# Autodesk Inventor assembly: main_assy
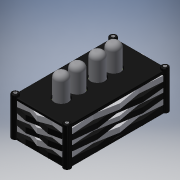
[picture p0: Inventor's stored thumbnail of the model, 180x180]
Saved by Autodesk Inventor 2017 (Build 210142000, 142)
## iProperties
Created: 2018-01-14
Part Number: main_assy
Document SubType Name: Assembly
Designer: Mitch
Author: Mitch
## Documents named in this file (26)
- E:\Youtube Channel\Pojects\Nixie Clock\Mech\main_assy.iam
- E:\Youtube Channel\Pojects\Nixie Clock\Mech\Clock Base.ipt
- E:\Youtube Channel\Pojects\Nixie Clock\Mech\PCB.ipt
- E:\Youtube Channel\Pojects\Nixie Clock\Mech\High_volt_pcb.ipt
- E:\Youtube Channel\Pojects\Nixie Clock\Mech\Case Top.ipt
- E:\Youtube Channel\Pojects\Nixie Clock\Mech\long_insert.ipt
- E:\Youtube Channel\Pojects\Nixie Clock\Mech\long_insert_inv.ipt
- E:\Youtube Channel\Pojects\Nixie Clock\Mech\Short_insert.ipt
- E:\Youtube Channel\Pojects\Nixie Clock\Mech\short_insert_invert.ipt
- E:\Youtube Channel\Pojects\Nixie Clock\Mech\long_insert_CPY.ipt
- E:\Youtube Channel\Pojects\Nixie Clock\Mech\long_insert_inv_CPY.ipt
- E:\Youtube Channel\Pojects\Nixie Clock\Mech\long_insert_CPY1.ipt
- E:\Youtube Channel\Pojects\Nixie Clock\Mech\long_insert_inv_CPY1.ipt
- E:\Youtube Channel\Pojects\Nixie Clock\Mech\Short_insert_CPY.ipt
- E:\Youtube Channel\Pojects\Nixie Clock\Mech\short_insert_invert_CPY.ipt
- E:\Youtube Channel\Pojects\Nixie Clock\Mech\Short_insert_CPY1.ipt
- E:\Youtube Channel\Pojects\Nixie Clock\Mech\short_insert_invert_CPY1.ipt
- E:\Youtube Channel\Pojects\Nixie Clock\Mech\Short_insert_CPY2.ipt
- E:\Youtube Channel\Pojects\Nixie Clock\Mech\short_insert_invert_CPY2.ipt
- E:\Youtube Channel\Pojects\Nixie Clock\Mech\Short_insert_CPY3.ipt
- E:\Youtube Channel\Pojects\Nixie Clock\Mech\short_insert_invert_CPY3.ipt
- E:\Youtube Channel\Pojects\Nixie Clock\Mech\back_plate.ipt
- E:\Youtube Channel\Pojects\Nixie Clock\Mech\91500A084_TYPE 316 SS FLAT HEAD PHILLIPS MACHINE SCREW.ipt
- E:\Youtube Channel\Pojects\Nixie Clock\Mech\Tactile switch Omron_B3F.iam
- E:\Youtube Channel\Pojects\Nixie Clock\Mech\CUI_PJ-002B.ipt
- E:\Youtube Channel\Pojects\Nixie Clock\Mech\push_buttons.ipt
## Components (31 placed, 25 different names)
1. Clock Base:1 — Mate:4, Mate:5, Mate:6, Mate:7, Mate:8, Mate:9, Mate:10, Mate:12, Mate:13, Mate:14, Mate:16, Mate:17, Mate:19, Mate:20, Mate:21, Mate:22, Mate:23, Mate:25, Mate:26, Mate:31, Mate:32, Mate:33, Mate:34, Mate:35, Mate:36, Mate:37, Mate:38, Mate:39, Mate:44, Mate:45, Mate:46, Mate:47, Mate:48, Mate:49, Mate:50, Mate:51, Mate:56, Mate:57, Mate:58, Mate:59, Mate:60, Mate:61, Mate:62, Mate:63, Mate:64, Mate:65, Mate:66, Flush:1, Mate:68, Mate:69, Mate:70, Mate:71, Mate:72
2. High_volt_pcb:1 — Mate:4, Mate:5, Mate:6
3. Case Top:1 — Mate:7, Flush:2, Flush:3, Flush:4, Flush:5
4. long_insert:1 — Mate:8, Mate:9, Mate:10, Mate:18
5. long_insert_inv:1 — Mate:18, Mate:19, Mate:20, Mate:27
6. Short_insert:1 — Mate:12, Mate:13, Mate:14, Mate:15
7. short_insert_invert:1 — Mate:15, Mate:16, Mate:17, Mate:40
8. Short_insert:2 — Mate:21, Mate:22, Mate:23, Mate:24
9. short_insert_invert:2 — Mate:24, Mate:25, Mate:26, Mate:52
10. long_insert_CPY:1 — Mate:27, Mate:28, Mate:31, Mate:32, Mate:39
11. long_insert_inv_CPY:1 — Mate:28, Mate:29, Mate:33, Mate:38
12. long_insert_CPY1:1 — Mate:29, Mate:30, Mate:35, Mate:37
13. long_insert_inv_CPY1:1 — Mate:30, Mate:34, Mate:36
14. Short_insert_CPY:1 — Mate:40, Mate:41, Mate:44, Mate:48
15. short_insert_invert_CPY:1 — Mate:41, Mate:42, Mate:45, Mate:49
16. Short_insert_CPY1:1 — Mate:42, Mate:43, Mate:46, Mate:50
17. short_insert_invert_CPY1:1 — Mate:43, Mate:47, Mate:51
18. Short_insert_CPY2:1 — Mate:52, Mate:53, Mate:56, Mate:60
19. short_insert_invert_CPY2:1 — Mate:53, Mate:54, Mate:57, Mate:61
20. Short_insert_CPY3:1 — Mate:54, Mate:55, Mate:58, Mate:62
21. short_insert_invert_CPY3:1 — Mate:55, Mate:59, Mate:63
22. back_plate:1 — Mate:64, Mate:65, Mate:66, Mate:67, Mate:78, Mate:79, Mate:80
23. PCB:1 — Mate:67, Flush:1, Mate:68, Mate:73, Mate:74, Mate:75, Flush:6, Flush:7, Mate:76, Mate:77, Flush:8, Flush:9
24. 91500A084_TYPE 316 SS FLAT HEAD PHILLIPS MACHINE SCREW:1 — Mate:69, Flush:4
25. 91500A084_TYPE 316 SS FLAT HEAD PHILLIPS MACHINE SCREW:2 — Mate:70, Flush:3
26. 91500A084_TYPE 316 SS FLAT HEAD PHILLIPS MACHINE SCREW:3 — Mate:72, Flush:5
27. 91500A084_TYPE 316 SS FLAT HEAD PHILLIPS MACHINE SCREW:4 — Mate:71, Flush:2
28. Tactile switch Omron_B3F:1 [sub-assembly] — Mate:74, Mate:77, Flush:8
29. Tactile switch Omron_B3F:2 [sub-assembly] — Mate:75, Mate:76, Flush:9
30. CUI_PJ-002B:1 — Mate:73, Flush:6, Flush:7
31. push_buttons:1 — Mate:78, Mate:79, Mate:80
## Relationships (85: Mate 76, Flush 9)
- Mate:4 (3.81 mm): Clock Base:1 ↔ High_volt_pcb:1
- Mate:5: Clock Base:1 ↔ High_volt_pcb:1
- Mate:6: Clock Base:1 ↔ High_volt_pcb:1
- Mate:7: Clock Base:1 ↔ Case Top:1
- Mate:8 (0.381 mm): Clock Base:1 ↔ long_insert:1
- Mate:9: Clock Base:1 ↔ long_insert:1
- Mate:10 (0.1778 mm): Clock Base:1 ↔ long_insert:1
- Mate:12: Clock Base:1 ↔ Short_insert:1
- Mate:13 (0.1778 mm): Clock Base:1 ↔ Short_insert:1
- Mate:14 (0.381 mm): Clock Base:1 ↔ Short_insert:1
- Mate:15: Short_insert:1 ↔ short_insert_invert:1
- Mate:16 (0.1778 mm): Clock Base:1 ↔ short_insert_invert:1
- Mate:17 (0.381 mm): Clock Base:1 ↔ short_insert_invert:1
- Mate:18: long_insert:1 ↔ long_insert_inv:1
- Mate:19 (0.1778 mm): Clock Base:1 ↔ long_insert_inv:1
- Mate:20 (0.381 mm): Clock Base:1 ↔ long_insert_inv:1
- Mate:21: Clock Base:1 ↔ Short_insert:2
- Mate:22 (0.1778 mm): Clock Base:1 ↔ Short_insert:2
- Mate:23 (0.381 mm): Clock Base:1 ↔ Short_insert:2
- Mate:24: Short_insert:2 ↔ short_insert_invert:2
- Mate:25 (0.1778 mm): Clock Base:1 ↔ short_insert_invert:2
- Mate:26 (0.381 mm): Clock Base:1 ↔ short_insert_invert:2
- Mate:27: long_insert_inv:1 ↔ long_insert_CPY:1
- Mate:28: long_insert_CPY:1 ↔ long_insert_inv_CPY:1
- Mate:29: long_insert_inv_CPY:1 ↔ long_insert_CPY1:1
- Mate:30: long_insert_CPY1:1 ↔ long_insert_inv_CPY1:1
- Mate:31 (0.1778 mm): Clock Base:1 ↔ long_insert_CPY:1
- Mate:32 (0.1778 mm): Clock Base:1 ↔ long_insert_CPY:1
- Mate:33 (0.1778 mm): Clock Base:1 ↔ long_insert_inv_CPY:1
- Mate:34 (0.1778 mm): Clock Base:1 ↔ long_insert_inv_CPY1:1
- Mate:35 (0.1778 mm): Clock Base:1 ↔ long_insert_CPY1:1
- Mate:36 (0.381 mm): Clock Base:1 ↔ long_insert_inv_CPY1:1
- Mate:37 (0.381 mm): Clock Base:1 ↔ long_insert_CPY1:1
- Mate:38 (0.381 mm): Clock Base:1 ↔ long_insert_inv_CPY:1
- Mate:39 (0.381 mm): Clock Base:1 ↔ long_insert_CPY:1
- Mate:40: short_insert_invert:1 ↔ Short_insert_CPY:1
- Mate:41: Short_insert_CPY:1 ↔ short_insert_invert_CPY:1
- Mate:42: short_insert_invert_CPY:1 ↔ Short_insert_CPY1:1
- Mate:43: Short_insert_CPY1:1 ↔ short_insert_invert_CPY1:1
- Mate:44 (0.1778 mm): Clock Base:1 ↔ Short_insert_CPY:1
- Mate:45 (0.1778 mm): Clock Base:1 ↔ short_insert_invert_CPY:1
- Mate:46 (0.1778 mm): Clock Base:1 ↔ Short_insert_CPY1:1
- Mate:47 (0.1778 mm): Clock Base:1 ↔ short_insert_invert_CPY1:1
- Mate:48 (0.381 mm): Clock Base:1 ↔ Short_insert_CPY:1
- Mate:49 (0.381 mm): Clock Base:1 ↔ short_insert_invert_CPY:1
- Mate:50 (0.381 mm): Clock Base:1 ↔ Short_insert_CPY1:1
- Mate:51 (0.381 mm): Clock Base:1 ↔ short_insert_invert_CPY1:1
- Mate:52: short_insert_invert:2 ↔ Short_insert_CPY2:1
- Mate:53: Short_insert_CPY2:1 ↔ short_insert_invert_CPY2:1
- Mate:54: short_insert_invert_CPY2:1 ↔ Short_insert_CPY3:1
- Mate:55: Short_insert_CPY3:1 ↔ short_insert_invert_CPY3:1
- Mate:56 (0.1778 mm): Clock Base:1 ↔ Short_insert_CPY2:1
- Mate:57 (0.1778 mm): Clock Base:1 ↔ short_insert_invert_CPY2:1
- Mate:58 (0.1778 mm): Clock Base:1 ↔ Short_insert_CPY3:1
- Mate:59 (0.1778 mm): Clock Base:1 ↔ short_insert_invert_CPY3:1
- Mate:60 (0.381 mm): Clock Base:1 ↔ Short_insert_CPY2:1
- Mate:61 (0.381 mm): Clock Base:1 ↔ short_insert_invert_CPY2:1
- Mate:62 (0.381 mm): Clock Base:1 ↔ Short_insert_CPY3:1
- Mate:63 (0.381 mm): Clock Base:1 ↔ short_insert_invert_CPY3:1
- Mate:64: Clock Base:1 ↔ back_plate:1
- Mate:65 (0.1778 mm): Clock Base:1 ↔ back_plate:1
- Mate:66 (0.381 mm): Clock Base:1 ↔ back_plate:1
- Mate:67: back_plate:1 ↔ PCB:1
- Flush:1 (13.97 mm): Clock Base:1 ↔ PCB:1
- Mate:68: Clock Base:1 ↔ PCB:1
- Mate:69: Clock Base:1 ↔ 91500A084_TYPE 316 SS FLAT HEAD PHILLIPS MACHINE SCREW:1
- Mate:70: Clock Base:1 ↔ 91500A084_TYPE 316 SS FLAT HEAD PHILLIPS MACHINE SCREW:2
- Mate:71: Clock Base:1 ↔ 91500A084_TYPE 316 SS FLAT HEAD PHILLIPS MACHINE SCREW:4
- Mate:72: Clock Base:1 ↔ 91500A084_TYPE 316 SS FLAT HEAD PHILLIPS MACHINE SCREW:3
- Flush:2: Case Top:1 ↔ 91500A084_TYPE 316 SS FLAT HEAD PHILLIPS MACHINE SCREW:4
- Flush:3: Case Top:1 ↔ 91500A084_TYPE 316 SS FLAT HEAD PHILLIPS MACHINE SCREW:2
- Flush:4: Case Top:1 ↔ 91500A084_TYPE 316 SS FLAT HEAD PHILLIPS MACHINE SCREW:1
- Flush:5: Case Top:1 ↔ 91500A084_TYPE 316 SS FLAT HEAD PHILLIPS MACHINE SCREW:3
- Mate:73: PCB:1 ↔ CUI_PJ-002B:1
- Mate:74: PCB:1 ↔ Tactile switch Omron_B3F:1
- Mate:75: PCB:1 ↔ Tactile switch Omron_B3F:2
- Flush:6: PCB:1 ↔ CUI_PJ-002B:1
- Flush:7 (6.35 mm): PCB:1 ↔ CUI_PJ-002B:1
- Mate:76 (-5.08 mm): PCB:1 ↔ Tactile switch Omron_B3F:2
- Mate:77 (-5.08 mm): PCB:1 ↔ Tactile switch Omron_B3F:1
- Flush:8 (52.8193 mm): PCB:1 ↔ Tactile switch Omron_B3F:1
- Flush:9 (64.2493 mm): PCB:1 ↔ Tactile switch Omron_B3F:2
- Mate:78: back_plate:1 ↔ push_buttons:1
- Mate:79: back_plate:1 ↔ push_buttons:1
- Mate:80: back_plate:1 ↔ push_buttons:1
